# Autodesk Inventor assembly: Assembly2
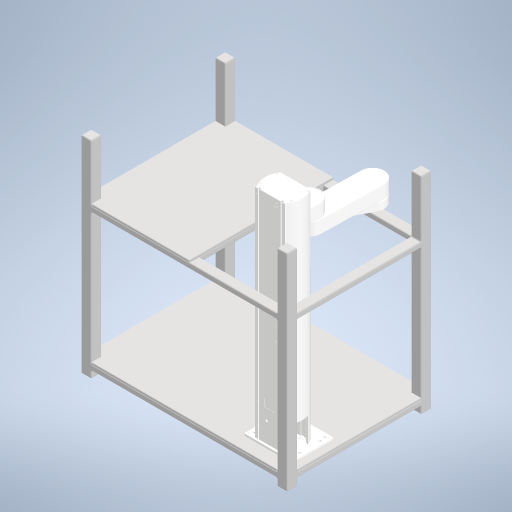
[picture p0: Inventor's stored thumbnail of the model, 512x512]
Saved by Autodesk Inventor 2023 (Build 270158000, 158)
## iProperties
Created: 2022-09-20
Part Number: Assembly2
Document SubType Name: Assembly
Designer: benni
Author: benni
## Documents named in this file (3)
- C:\Users\benni\Documents\Studium\7. Semester\Industrial Robotics\Assignment 2\@PF3400\CAD\Assembly2.iam
- C:\Users\benni\Documents\Studium\7. Semester\Industrial Robotics\Assignment 2\@PF3400\CAD\Assembly1.iam
- C:\Users\benni\Documents\Studium\7. Semester\Industrial Robotics\Assignment 2\@Objects\Table.ipt
## Components (2 placed, 2 different names)
1. Assembly1:1 [sub-assembly] — Mate:1
2. Table:1 — Mate:1
## Relationships (1: Mate 1)
- Mate:1: Assembly1:1 ↔ Table:1
